# Autodesk Inventor assembly: Dai
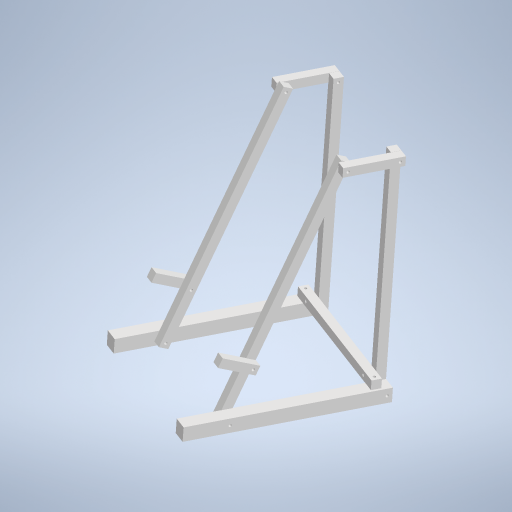
[picture p0: Inventor's stored thumbnail of the model, 512x512]
Saved by Autodesk Inventor 2023 (Build 270158000, 158)
## iProperties
Created: 2022-10-24
Part Number: Dai
Document SubType Name: Assembly
Designer: banru
Author: banru
## Documents named in this file (7)
- C:\Users\banru\Documents\workspace\Contactless\Inventor\Dai\Dai.iam
- C:\Users\banru\Documents\workspace\Contactless\Inventor\Dai\Dai.ipt
- C:\Users\banru\Documents\workspace\Contactless\Inventor\Dai\Naname.ipt
- C:\Users\banru\Documents\workspace\Contactless\Inventor\Dai\Tate.ipt
- C:\Users\banru\Documents\workspace\Contactless\Inventor\Dai\DaiUe.ipt
- C:\Users\banru\Documents\workspace\Contactless\Inventor\Dai\Soko.ipt
- C:\Users\banru\Documents\workspace\Contactless\Inventor\Dai\Shita.ipt
## Components (11 placed, 6 different names)
1. Dai:1 — 挿入:1, 挿入:2, フラッシュ:1, 挿入:6
2. Naname:1 — 挿入:2, 挿入:4, 挿入:5, フラッシュ:2
3. Tate:1 — 挿入:1, フラッシュ:1, 挿入:3, 挿入:16
4. DaiUe:1 — 挿入:3, 挿入:4
5. Soko:1 — 挿入:5, フラッシュ:2
6. Shita:1 — 挿入:6, 挿入:7, 挿入:16, 挿入:17
7. Dai:2 — 挿入:7, 挿入:8, 挿入:9, フラッシュ:4
8. Tate:2 — 挿入:8, 挿入:13, フラッシュ:4, 挿入:17
9. Naname:2 — 挿入:9, フラッシュ:3, 挿入:15, 挿入:18
10. DaiUe:2 — 挿入:13, 挿入:18
11. Soko:2 — フラッシュ:3, 挿入:15
## Relationships (18: Insert 14, Flush 4)
- 挿入:1 [Insert]: Dai:1 ↔ Tate:1
- 挿入:2 [Insert]: Dai:1 ↔ Naname:1
- フラッシュ:1 [Flush]: Dai:1 ↔ Tate:1
- 挿入:3 [Insert]: Tate:1 ↔ DaiUe:1
- 挿入:4 [Insert]: Naname:1 ↔ DaiUe:1
- 挿入:5 [Insert]: Naname:1 ↔ Soko:1
- フラッシュ:2 [Flush]: Naname:1 ↔ Soko:1
- 挿入:6 [Insert]: Dai:1 ↔ Shita:1
- 挿入:7 [Insert]: Shita:1 ↔ Dai:2
- 挿入:8 [Insert]: Dai:2 ↔ Tate:2
- 挿入:9 [Insert]: Dai:2 ↔ Naname:2
- フラッシュ:3 [Flush]: Naname:2 ↔ Soko:2
- 挿入:13 [Insert]: Tate:2 ↔ DaiUe:2
- 挿入:15 [Insert]: Naname:2 ↔ Soko:2
- 挿入:16 [Insert]: Tate:1 ↔ Shita:1
- フラッシュ:4 [Flush]: Dai:2 ↔ Tate:2
- 挿入:17 [Insert]: Shita:1 ↔ Tate:2
- 挿入:18 [Insert]: Naname:2 ↔ DaiUe:2
